# Autodesk Inventor assembly: Projeto - Contrapeso
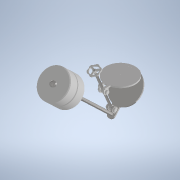
[picture p0: Inventor's stored thumbnail of the model, 180x180]
Saved by Autodesk Inventor 2021 (Build 250183000, 183)
## iProperties
Created: 2021-08-26
Part Number: Projeto - Contrapeso
Document SubType Name: Assembly
Designer: guilh
Author: guilh
## Documents named in this file (11)
- D:\Documentos\Astronomia\Projeto Equatorial\Counterwheight System\Counterweight System Project.iam
- D:\Documentos\Astronomia\Projeto Equatorial\Counterwheight System\Telescope Base - Equatorial.ipt
- D:\Documentos\Astronomia\Projeto Equatorial\Counterwheight System\Butterfly.ipt
- D:\Documentos\Astronomia\Projeto Equatorial\Counterwheight System\Angle Control.ipt
- D:\Documentos\Astronomia\Projeto Equatorial\Counterwheight System\Hinge.ipt
- D:\Documentos\Astronomia\Projeto Equatorial\Counterwheight System\Platform Pin.ipt
- D:\Documentos\Astronomia\Projeto Equatorial\Counterwheight System\Hinge Pin.ipt
- D:\Documentos\Astronomia\Projeto Equatorial\Counterwheight System\Tripod Base - Equatorial.ipt
- D:\Documentos\Astronomia\Projeto Equatorial\Counterwheight System\Counterweight Rod.ipt
- D:\Documentos\Astronomia\Projeto Equatorial\Counterwheight System\Peso.ipt
- D:\Documentos\Astronomia\Projeto Equatorial\Counterwheight System\Telescope Base Pin.ipt
## Components (12 placed, 10 different names)
1. Tripod Base - Equatorial:1 — Mate:15, Insert:7, Insert:8, Mate:16, Flush:4
2. Telescope Base - Equatorial:1 — Mate:6, Insert:5, Insert:6, Flush:3, Mate:18, Insert:9
3. Butterfly:1 — Mate:1, Mate:2, Flush:1
4. Angle Control:1 — Mate:1, Mate:2, Flush:1, Mate:7, Insert:10
5. Hinge:1 — Insert:1, Mate:6, Insert:5, Insert:6
6. Hinge:2 — Insert:2, Mate:15, Insert:7, Insert:8
7. Hinge Pin:1 — Insert:1, Insert:2
8. Platform Pin:2 — Mate:7, Mate:16, Flush:4
9. Counterweight Rod:1 — Flush:3, Mate:10, Mate:11, Mate:12, Mate:18
10. Peso:1 — Mate:11, Mate:12, Mate:13
11. Peso:2 — Mate:10, Mate:13
12. Telescope Base Pin:1 — Insert:9, Insert:10
## Relationships (22: Mate 11, Insert 8, Flush 3)
- Mate:1: Butterfly:1 ↔ Angle Control:1
- Mate:2: Butterfly:1 ↔ Angle Control:1
- Flush:1: Butterfly:1 ↔ Angle Control:1
- Insert:1: Hinge:1 ↔ Hinge Pin:1
- Insert:2: Hinge:2 ↔ Hinge Pin:1
- Mate:6: Telescope Base - Equatorial:1 ↔ Hinge:1
- Mate:7: Angle Control:1 ↔ Platform Pin:2
- Insert:5: Telescope Base - Equatorial:1 ↔ Hinge:1
- Insert:6: Telescope Base - Equatorial:1 ↔ Hinge:1
- Flush:3: Telescope Base - Equatorial:1 ↔ Counterweight Rod:1
- Mate:10: Counterweight Rod:1 ↔ Peso:2
- Mate:11: Counterweight Rod:1 ↔ Peso:1
- Mate:12: Counterweight Rod:1 ↔ Peso:1
- Mate:13: Peso:1 ↔ Peso:2
- Mate:15: Tripod Base - Equatorial:1 ↔ Hinge:2
- Insert:7: Tripod Base - Equatorial:1 ↔ Hinge:2
- Insert:8: Tripod Base - Equatorial:1 ↔ Hinge:2
- Mate:16: Tripod Base - Equatorial:1 ↔ Platform Pin:2
- Flush:4 (-10 mm): Tripod Base - Equatorial:1 ↔ Platform Pin:2
- Mate:18: Telescope Base - Equatorial:1 ↔ Counterweight Rod:1
- Insert:9 (-8 mm): Telescope Base - Equatorial:1 ↔ Telescope Base Pin:1
- Insert:10: Angle Control:1 ↔ Telescope Base Pin:1
